# Autodesk Inventor assembly: full_assembly
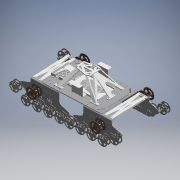
[picture p0: Inventor's stored thumbnail of the model, 180x180]
Saved by Autodesk Inventor 2019.4 (Build 234330000, 330)
## iProperties
Part Number: full_assembly
Document SubType Name: Assembly
Designer: Jorge
Author: Jorge
## Documents named in this file (8)
- D:\TFG\dev\hardware\ROVER\full_assembly.iam
- D:\TFG\dev\hardware\ROVER\platform.iam
- D:\TFG\dev\hardware\ROVER\LIDAR_support.ipt
- D:\TFG\dev\hardware\ROVER\PCB_deck.ipt
- D:\TFG\dev\hardware\ROVER\Deck.ipt
- D:\TFG\dev\hardware\ROVER\battery-strap casing.ipt
- D:\TFG\dev\hardware\ROVER\battery-strap -under.ipt
- D:\TFG\dev\hardware\ROVER\stabilizer.ipt
## Components (10 placed, 7 different names)
1. platform:1 [sub-assembly] — Mate:1, Mate:2, Angle:1, Mate:3, Mate:4, Angle:2, Mate:5, Angle:3, Flush:1, Mate:6, Mate:7, Mate:8, Mate:9, Angle:4, Angle:5, Mate:10, Mate:11, Angle:6, Angle:7, Mate:14, Mate:15, Mate:16, Mate:17, Mate:18, Mate:19, Mate:20, Mate:21
2. LIDAR_support:1 — Mate:1, Mate:2, Angle:1
3. PCB_deck:1 — Mate:3, Mate:4, Angle:2
4. Deck:1 — Mate:5, Angle:3, Flush:1
5. battery-strap casing:1 — Mate:7, Mate:9, Angle:5
6. battery-strap casing:2 — Mate:6, Mate:8, Angle:4
7. battery-strap -under:1 — Mate:10, Angle:7, Mate:14
8. battery-strap -under:2 — Mate:11, Angle:6, Mate:15
9. stabilizer:1 — Mate:16, Mate:17, Mate:18
10. stabilizer:2 — Mate:19, Mate:20, Mate:21
## Relationships (27: Mate 19, Angle 7, Flush 1)
- Mate:1: platform:1 ↔ LIDAR_support:1
- Mate:2: platform:1 ↔ LIDAR_support:1
- Angle:1 (0 deg): platform:1 ↔ LIDAR_support:1
- Mate:3: platform:1 ↔ PCB_deck:1
- Mate:4 (1.42 mm): platform:1 ↔ PCB_deck:1
- Angle:2 (0 deg): platform:1 ↔ PCB_deck:1
- Mate:5: platform:1 ↔ Deck:1
- Angle:3 (0 deg): platform:1 ↔ Deck:1
- Flush:1 (-5 mm): platform:1 ↔ Deck:1
- Mate:6: platform:1 ↔ battery-strap casing:2
- Mate:7: platform:1 ↔ battery-strap casing:1
- Mate:8: platform:1 ↔ battery-strap casing:2
- Mate:9: platform:1 ↔ battery-strap casing:1
- Angle:4 (180 deg): platform:1 ↔ battery-strap casing:2
- Angle:5 (180 deg): platform:1 ↔ battery-strap casing:1
- Mate:10: platform:1 ↔ battery-strap -under:1
- Mate:11: platform:1 ↔ battery-strap -under:2
- Angle:6 (180 deg): platform:1 ↔ battery-strap -under:2
- Angle:7 (180 deg): platform:1 ↔ battery-strap -under:1
- Mate:14: platform:1 ↔ battery-strap -under:1
- Mate:15: platform:1 ↔ battery-strap -under:2
- Mate:16: platform:1 ↔ stabilizer:1
- Mate:17: platform:1 ↔ stabilizer:1
- Mate:18: platform:1 ↔ stabilizer:1
- Mate:19: platform:1 ↔ stabilizer:2
- Mate:20: platform:1 ↔ stabilizer:2
- Mate:21: platform:1 ↔ stabilizer:2
